# Autodesk Inventor assembly: fc16-044
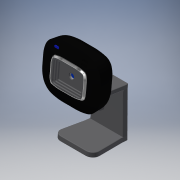
[picture p0: Inventor's stored thumbnail of the model, 180x180]
Saved by Autodesk Inventor 2017.1 (Build 211199000, 199)
## iProperties
Category: Electronics
Company: Autodesk Inc.
Created: 2016-12-16
Part Number: fc16-044
Document SubType Name: Assembly
Designer: Autodesk Inc.
Catalog Web Link: http://www.microsoft.com/hardware/en-ca/p/lifecam-hd-3000
Vendor: Microsoft Inc.
Author: Autodesk Inc.
Keywords: FIRSTChoice
## Documents named in this file (3)
- D:\FIRST\FIRST KOP 2017\FIRST FirstChoice 2017\fc17-048_Camera.iam
- D:\FIRST\FIRST KOP 2017\FIRST FirstChoice 2017\Parts\CS_Camera_HD3000.ipt
- D:\FIRST\FIRST KOP 2017\FIRST FirstChoice 2017\Parts\CS_Camera_HD3000_Base_01.ipt
## Components (2 placed, 2 different names)
1. CS_Camera_HD3000:1 — Mate:1, Mate:2
2. CS_Camera_HD3000_Base_01:1 — Mate:1, Mate:2
## Relationships (2: Mate 2)
- Mate:1: CS_Camera_HD3000:1 ↔ CS_Camera_HD3000_Base_01:1
- Mate:2: CS_Camera_HD3000:1 ↔ CS_Camera_HD3000_Base_01:1
